# Autodesk Inventor assembly: 04-0001
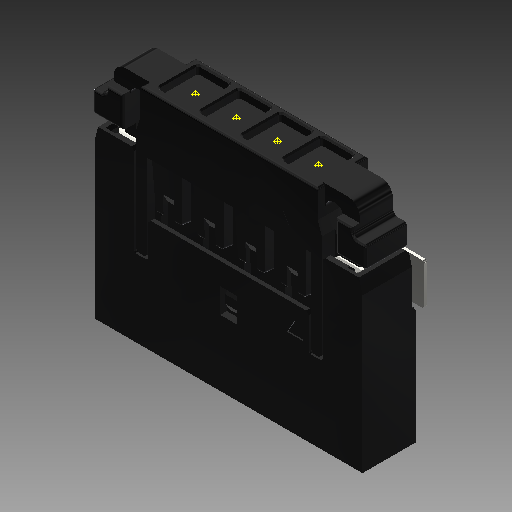
[picture p0: Inventor's stored thumbnail of the model, 512x512]
Saved by Autodesk Inventor 2018 (Build 220112000, 112)
## iProperties
Created: 2019-09-21
Part Number: 04-0001
Document SubType Name: Assembly
Designer: Bradley
Author: Bradley
## Documents named in this file (3)
- C:\Users\Bradley\Documents\GitHub\Resources\SupplierDocuments\04 - Connectors SMT\04-0001\04-0001.iam
- C:\Users\Bradley\Documents\GitHub\Resources\SupplierDocuments\04 - Connectors SMT\04-0001\04-0001.ipt
- C:\Users\Bradley\Documents\GitHub\Resources\SupplierDocuments\04 - Connectors SMT\04-0001P\04-0001P.ipt
## Components (2 placed, 2 different names)
1. 04-0001:1 — Flush:1, Mate:2, Mate:3
2. 04-0001P:1 — Flush:1, Mate:2, Mate:3
## Relationships (3: Mate 2, Flush 1)
- Flush:1: 04-0001:1 ↔ 04-0001P:1
- Mate:2: 04-0001:1 ↔ 04-0001P:1
- Mate:3: 04-0001:1 ↔ 04-0001P:1
